# Autodesk Inventor assembly: CAJA
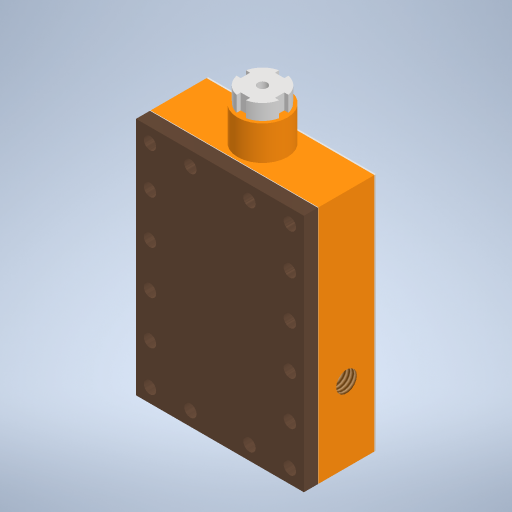
[picture p0: Inventor's stored thumbnail of the model, 512x512]
Saved by Autodesk Inventor 2024.2 (Build 282272000, 272)
## iProperties
Created: 2024-11-02
Part Number: CAJA
Document SubType Name: Assembly
Designer: melim
Author: melim
## Documents named in this file (6)
- C:\Users\melim\OneDrive\Desktop\PIEZAS_MELISSA\CAJA.iam
- C:\Users\melim\OneDrive\Desktop\PIEZAS_MELISSA\HUDSON-1-32.ipt
- C:\Users\melim\OneDrive\Desktop\PIEZAS_MELISSA\HUDSON-1-34.ipt
- C:\Users\melim\OneDrive\Desktop\PIEZAS_MELISSA\HUDSON-1-35.ipt
- C:\Users\melim\OneDrive\Desktop\PIEZAS_MELISSA\HUDSON-1-33.ipt
- C:\Users\melim\OneDrive\Desktop\PIEZAS_MELISSA\HUDSON-1-36.ipt
## Components (5 placed, 5 different names)
1. HUDSON-1-32:1 — Mate:1, Mate:2, Mate:3, Mate:4, Mate:5, Mate:7, Mate:8, Mate:9, Mate:10, Mate:11, Mate:12, Mate:13, Mate:14, Mate:15
2. HUDSON-1-34:1 — Mate:1, Mate:2, Mate:3, Mate:4, Mate:6
3. HUDSON-1-35:1 — Mate:5, Mate:6, Mate:7, Mate:8
4. HUDSON-1-33:1 — Mate:9, Mate:10, Mate:11, Mate:12, Mate:13
5. HUDSON-1-36:1 — Mate:14, Mate:15
## Relationships (15: Mate 15)
- Mate:1: HUDSON-1-32:1 ↔ HUDSON-1-34:1
- Mate:2: HUDSON-1-32:1 ↔ HUDSON-1-34:1
- Mate:3: HUDSON-1-32:1 ↔ HUDSON-1-34:1
- Mate:4: HUDSON-1-32:1 ↔ HUDSON-1-34:1
- Mate:5: HUDSON-1-32:1 ↔ HUDSON-1-35:1
- Mate:6: HUDSON-1-34:1 ↔ HUDSON-1-35:1
- Mate:7: HUDSON-1-32:1 ↔ HUDSON-1-35:1
- Mate:8: HUDSON-1-32:1 ↔ HUDSON-1-35:1
- Mate:9: HUDSON-1-32:1 ↔ HUDSON-1-33:1
- Mate:10: HUDSON-1-32:1 ↔ HUDSON-1-33:1
- Mate:11: HUDSON-1-32:1 ↔ HUDSON-1-33:1
- Mate:12: HUDSON-1-32:1 ↔ HUDSON-1-33:1
- Mate:13: HUDSON-1-32:1 ↔ HUDSON-1-33:1
- Mate:14: HUDSON-1-32:1 ↔ HUDSON-1-36:1
- Mate:15: HUDSON-1-32:1 ↔ HUDSON-1-36:1
